# Autodesk Inventor assembly: Leg_Link_Flame_8
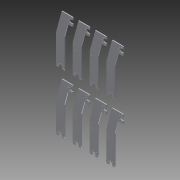
[picture p0: Inventor's stored thumbnail of the model, 180x180]
Saved by Autodesk Inventor 2013 (Build 170138000, 138)
## iProperties
Created: 2014-04-26
Part Number: Leg_Link_Flame_8
Document SubType Name: Assembly
Designer: andou
Author: andou
## Documents named in this file (2)
- C:\Users\andou\Documents\GitHub\Robotics-Project\design\RoboticsProject\project_4\cnc_data\Leg_Link_Flame_8.iam
- C:\Users\andou\Documents\GitHub\Robotics-Project\design\RoboticsProject\project_4\cnc_data\Leg_Link_Flame_4.iam
## Components (2 placed, 1 different names)
1. Leg_Link_Flame_4:1 [sub-assembly]
2. Leg_Link_Flame_4:2 [sub-assembly]
## Component patterns: (2 elements, first: Leg_Link_Flame_4:1)
